# Autodesk Inventor assembly: Motedius_QR-500
(part 2 of 2)
- [Mate]: Motedius_Gelenkfuß_10_PA_M6x60:2 ↔ DIN 125-1 A A 6,4:19
- [Mate]: Motedius_Gelenkfuß_10_PA_M6x60:2 ↔ DIN 125-1 A A 6,4:19
- Einfügen:30 [Insert] (5.5 mm): Motedius_20x20_B-Type_Slot-6_500:2 ↔ DIN 125-1 A A 6,4:19
- [Mate]: Motedius_Gelenkfuß_10_PA_M6x60:3 ↔ DIN 125-1 A A 6,4:20
- [Mate]: Motedius_Gelenkfuß_10_PA_M6x60:3 ↔ DIN 125-1 A A 6,4:20
- [Mate]: Motedius_Gelenkfuß_10_PA_M6x60:4 ↔ DIN 125-1 A A 6,4:21
- [Mate]: Motedius_Gelenkfuß_10_PA_M6x60:4 ↔ DIN 125-1 A A 6,4:21
- Einfügen:31 [Insert] (5.5 mm): Motedius_20x20_B-Type_Slot-6_500:4 ↔ DIN 125-1 A A 6,4:20
- Einfügen:32 [Insert] (5.5 mm): Motedius_20x20_B-Type_Slot-6_500:2 ↔ DIN 125-1 A A 6,4:21
- Passend:88 [Mate]: Motedius_Gelenkfuß_10_PA_M6x60:2 ↔ DIN 125-1 A A 6,4:22
- Passend:89 [Mate]: Motedius_20x20_B-Type_Slot-6_500:1 ↔ DIN 125-1 A A 6,4:22
- Passend:90 [Mate]: Motedius_Gelenkfuß_10_PA_M6x60:4 ↔ DIN 125-1 A A 6,4:23
- Passend:91 [Mate]: Motedius_20x20_B-Type_Slot-6_500:3 ↔ DIN 125-1 A A 6,4:23
- Passend:92 [Mate]: Motedius_Gelenkfuß_10_PA_M6x60:3 ↔ DIN 125-1 A A 6,4:24
- Passend:93 [Mate]: Motedius_20x20_B-Type_Slot-6_500:3 ↔ DIN 125-1 A A 6,4:24
- Passend:94 [Mate]: Motedius_Gelenkfuß_10_PA_M6x60:2 ↔ DIN 934 - ersetzt durch DIN EN 24032/28673/28674 M6:10
- Passend:95 [Mate]: DIN 125-1 A A 6,4:22 ↔ DIN 934 - ersetzt durch DIN EN 24032/28673/28674 M6:10
- Passend:96 [Mate]: Motedius_Gelenkfuß_10_PA_M6x60:4 ↔ DIN 934 - ersetzt durch DIN EN 24032/28673/28674 M6:11
- Passend:97 [Mate]: DIN 125-1 A A 6,4:23 ↔ DIN 934 - ersetzt durch DIN EN 24032/28673/28674 M6:11
- Passend:98 [Mate]: Motedius_Gelenkfuß_10_PA_M6x60:3 ↔ DIN 934 - ersetzt durch DIN EN 24032/28673/28674 M6:12
- Passend:99 [Mate]: DIN 125-1 A A 6,4:24 ↔ DIN 934 - ersetzt durch DIN EN 24032/28673/28674 M6:12
- Passend:135 [Mate]: Motedius_20x20_B-Type_Slot-6_600:1 ↔ Motedius_20x20_B-Type_Slot-6_290:1
- Fluchtend:23 [Flush]: Motedius_20x20_B-Type_Slot-6_600:1 ↔ Motedius_20x20_B-Type_Slot-6_290:1
- Fluchtend:24 [Flush] (290 mm): Motedius_20x20_B-Type_Slot-6_600:1 ↔ Motedius_20x20_B-Type_Slot-6_290:1
- Fluchtend:25 [Flush]: Motedius_20x20_B-Type_Slot-6_600:1 ↔ Motedius_20x20_B-Type_Slot-6_290:2
- Passend:136 [Mate]: Motedius_20x20_B-Type_Slot-6_600:1 ↔ Motedius_20x20_B-Type_Slot-6_290:2
- Fluchtend:26 [Flush] (290 mm): Motedius_20x20_B-Type_Slot-6_600:1 ↔ Motedius_20x20_B-Type_Slot-6_290:2
- Passend:137 [Mate] (30 mm): Motedius_20x20_B-Type_Slot-6_500:3 ↔ Motedius_20x20_B-Type_Slot-6_600:1
- Fluchtend:27 [Flush] (1 mm): Motedius_20x20_B-Type_Slot-6_600:1 ↔ Motedis_Winkel:9
- Passend:138 [Mate]: Motedius_20x20_B-Type_Slot-6_600:1 ↔ Motedis_Winkel:9
- Passend:139 [Mate]: Motedius_20x20_B-Type_Slot-6_290:2 ↔ Motedis_Winkel:9
- Passend:140 [Mate]: Motedius_20x20_B-Type_Slot-6_290:1 ↔ Motedis_Winkel:10
- Passend:141 [Mate]: Motedius_20x20_B-Type_Slot-6_600:1 ↔ Motedis_Winkel:10
- Passend:142 [Mate]: Motedius_20x20_B-Type_Slot-6_600:1 ↔ Motedis_Winkel:11
- Passend:143 [Mate]: Motedius_20x20_B-Type_Slot-6_290:2 ↔ Motedis_Winkel:11
- Fluchtend:28 [Flush] (1 mm): Motedius_20x20_B-Type_Slot-6_290:2 ↔ Motedis_Winkel:11
- Passend:144 [Mate]: Motedius_20x20_B-Type_Slot-6_600:1 ↔ Motedis_Winkel:12
- Passend:145 [Mate]: Motedius_20x20_B-Type_Slot-6_290:1 ↔ Motedis_Winkel:12
- Fluchtend:29 [Flush] (1 mm): Motedius_20x20_B-Type_Slot-6_600:1 ↔ Motedis_Winkel:12
- Fluchtend:31 [Flush] (202.07 mm): Motedius_20x20_B-Type_Slot-6_500:4 ↔ Motedis_Winkel:10
- Passend:159 [Mate] (1.2 mm): Motedius_20x20_B-Type_Slot-6_500_MIR:3 ↔ Mauro_Wagen_QR_version:5
- Passend:160 [Mate] (4.45 mm): Motedius_20x20_B-Type_Slot-6_500_MIR:3 ↔ Mauro_Wagen_QR_version:5
- Passend:161 [Mate] (1.2 mm): Motedius_20x20_B-Type_Slot-6_500_MIR:4 ↔ Mauro_Wagen_QR_version:6
- Passend:162 [Mate] (4.45 mm): Motedius_20x20_B-Type_Slot-6_500_MIR:4 ↔ Mauro_Wagen_QR_version:6
- Passend:163 [Mate] (1.2 mm): Motedius_20x20_B-Type_Slot-6_500_MIR:1 ↔ Mauro_Wagen_QR_version:8
- Passend:164 [Mate] (4.45 mm): Motedius_20x20_B-Type_Slot-6_500_MIR:1 ↔ Mauro_Wagen_QR_version:8
- Passend:165 [Mate] (1.2 mm): Motedius_20x20_B-Type_Slot-6_500_MIR:2 ↔ Mauro_Wagen_QR_version:7
- Passend:166 [Mate] (4.45 mm): Motedius_20x20_B-Type_Slot-6_500_MIR:2 ↔ Mauro_Wagen_QR_version:7
- Fluchtend:32 [Flush]: Mauro_Wagen_QR_version:6 ↔ Mauro_Wagen_QR_version:7
- Fluchtend:33 [Flush]: Mauro_Wagen_QR_version:5 ↔ Mauro_Wagen_QR_version:8
- Einfügen:47 [Insert] (-3 mm): Mauro_Wagen_QR_version:8 ↔ 10mm_Alu_Linearwelle_500mm:1
- Einfügen:48 [Insert] (-3 mm): Mauro_Wagen_QR_version:7 ↔ 10mm_Alu_Linearwelle_500mm:2
- Einfügen:49 [Insert]: Lagerblock_Lm10UU:1 ↔ Linearlager_LM10UU:2
- Einfügen:50 [Insert]: Lagerblock_Lm10UU:1 ↔ Linearlager_LM10UU:1
- Einfügen:51 [Insert] (-200 mm): 10mm_Alu_Linearwelle_500mm:2 ↔ Lagerblock_Lm10UU:1
- Einfügen:52 [Insert] (220 mm): 10mm_Alu_Linearwelle_500mm:1 ↔ Lagerblock_Lm10UU:1
- [Insert] (5.5 mm): Motedius_20x20_B-Type_Slot-6_500:6 ↔ QR_Rahmenschraube_oben_M6x80:2
- [Insert] (5.5 mm): Motedius_20x20_B-Type_Slot-6_500:6 ↔ QR_Rahmenschraube_oben_M6x80:3
- [Insert] (5.5 mm): Motedius_20x20_B-Type_Slot-6_500:5 ↔ QR_Rahmenschraube_oben_M6x80:4
- [Insert] (5.5 mm): Motedius_20x20_B-Type_Slot-6_500:5 ↔ QR_Rahmenschraube_oben_M6x80:5
- [Insert] (5.5 mm): Motedius_20x20_B-Type_Slot-6_500:7 ↔ QR_Rahmenschraube_oben_M6x80:6
- [Insert] (5.5 mm): Motedius_20x20_B-Type_Slot-6_500:7 ↔ QR_Rahmenschraube_oben_M6x80:1
- [Insert] (5.5 mm): Motedius_20x20_B-Type_Slot-6_500:8 ↔ QR_Rahmenschraube_oben_M6x80:7
- [Insert] (5.5 mm): Motedius_20x20_B-Type_Slot-6_500:8 ↔ QR_Rahmenschraube_oben_M6x80:8
- Passend:169 [Mate]: DIN 84 - ersetzt durch DIN EN ISO 1207 M5 x 30:1 ↔ DIN 934 - ersetzt durch DIN EN 24032/28673/28674 M5:2
- Einfügen:65 [Insert] (1 mm): Nema17_Schrittmotor:4 ↔ GT2_20tooth:1
- Einfügen:66 [Insert] (1 mm): Nema17_Schrittmotor:1 ↔ GT2_20tooth:2
- Einfügen:67 [Insert] (1 mm): Nema17_Schrittmotor:2 ↔ GT2_20tooth:3
- Einfügen:68 [Insert] (1 mm): Nema17_Schrittmotor:3 ↔ GT2_20tooth:4
- [Insert] (5.5 mm): Motedius_20x20_B-Type_Slot-6_500:7 ↔ QR_Ramenschraube_unten_M6x60:1
- Einfügen:71 [Insert] (5.5 mm): Motedius_20x20_B-Type_Slot-6_500:5 ↔ QR_Rahmenschraube_oben_M6x80:8
- Einfügen:72 [Insert] (5.5 mm): Motedius_20x20_B-Type_Slot-6_500:5 ↔ QR_Rahmenschraube_oben_M6x80:3
- Einfügen:73 [Insert] (5.5 mm): Motedius_20x20_B-Type_Slot-6_500:8 ↔ QR_Rahmenschraube_oben_M6x80:4
- Einfügen:74 [Insert] (5.5 mm): Motedius_20x20_B-Type_Slot-6_500:8 ↔ QR_Rahmenschraube_oben_M6x80:6
- Einfügen:75 [Insert] (5.5 mm): Motedius_20x20_B-Type_Slot-6_500:7 ↔ QR_Rahmenschraube_oben_M6x80:2
- Einfügen:76 [Insert] (5.5 mm): Motedius_20x20_B-Type_Slot-6_500:6 ↔ QR_Rahmenschraube_oben_M6x80:7
- Einfügen:77 [Insert] (5.5 mm): Motedius_20x20_B-Type_Slot-6_500:6 ↔ QR_Rahmenschraube_oben_M6x80:5
- Einfügen:78 [Insert] (5.5 mm): Motedius_20x20_B-Type_Slot-6_500:7 ↔ QR_Ramenschraube_unten_M6x60:2
- Einfügen:79 [Insert] (5.5 mm): Motedius_20x20_B-Type_Slot-6_500:6 ↔ QR_Ramenschraube_unten_M6x60:4
- Einfügen:80 [Insert] (5.5 mm): Motedius_20x20_B-Type_Slot-6_500:6 ↔ QR_Ramenschraube_unten_M6x60:3
- Einfügen:81 [Insert]: QR_Ramenschraube_unten_M6x60:4 ↔ DIN 9021 6,4:1
- Einfügen:82 [Insert]: DIN 9021 6,4:1 ↔ Distanzscheibe_6x10x0,5mm:1
- Einfügen:83 [Insert]: Seilrolle:1 ↔ Distanzscheibe_6x10x0,5mm:1
- Einfügen:84 [Insert]: Seilrolle:1 ↔ Distanzscheibe_6x10x0,5mm:2
- Einfügen:85 [Insert]: DIN 9021 6,4:2 ↔ Distanzscheibe_6x10x0,5mm:2
- Einfügen:86 [Insert] (5.5 mm): Motedius_20x20_B-Type_Slot-6_500:5 ↔ QR_Ramenschraube_unten_M6x60:6
- Einfügen:87 [Insert] (5.5 mm): Motedius_20x20_B-Type_Slot-6_500:5 ↔ QR_Ramenschraube_unten_M6x60:5
- Einfügen:88 [Insert] (5.5 mm): Motedius_20x20_B-Type_Slot-6_500:8 ↔ QR_Ramenschraube_unten_M6x60:8
- Einfügen:89 [Insert] (5.5 mm): Motedius_20x20_B-Type_Slot-6_500:8 ↔ QR_Ramenschraube_unten_M6x60:7
- [Insert]: Nema17_Schrittmotor:5 ↔ Nema17_Montageplatte_Z-Achse:1
- [Tangent]: Nema17_Schrittmotor:5 ↔ Nema17_Montageplatte_Z-Achse:1
- [Insert] (3 mm): Nema17_Schrittmotor:5 ↔ DIN 84 - ersetzt durch DIN EN ISO 1207 M3 x 6:17
- [Insert] (3 mm): Nema17_Schrittmotor:5 ↔ DIN 84 - ersetzt durch DIN EN ISO 1207 M3 x 6:19
- [Insert] (3 mm): Nema17_Schrittmotor:5 ↔ DIN 84 - ersetzt durch DIN EN ISO 1207 M3 x 6:20
- [Insert] (3 mm): Nema17_Schrittmotor:5 ↔ DIN 84 - ersetzt durch DIN EN ISO 1207 M3 x 6:18
- Passend:175 [Mate] (2.4 mm): Motedius_20x20_B-Type_Slot-6_500_MIR:4 ↔ Nema17_Montageplatte_Z-Achse:1
- Fluchtend:34 [Flush]: Motedius_20x20_B-Type_Slot-6_500_MIR:4 ↔ Nema17_Montageplatte_Z-Achse:1
- Fluchtend:35 [Flush] (45 mm): Motedius_20x20_B-Type_Slot-6_500_MIR:4 ↔ Nema17_Montageplatte_Z-Achse:1
- Einfügen:95 [Insert]: Nema17_Montageplatte_Z-Achse:1 ↔ DIN 9021 5,3:1
- Einfügen:96 [Insert]: DIN 9021 5,3:1 ↔ DIN 9021 5,3:2
- Einfügen:97 [Insert]: Nema17_Montageplatte_Z-Achse:1 ↔ DIN 9021 5,3:4
- Einfügen:98 [Insert]: DIN 9021 5,3:3 ↔ DIN 9021 5,3:4
- Einfügen:99 [Insert] (-8 mm): Nema17_Schrittmotor:5 ↔ Wellenkupplung5-8mm:1
- Einfügen:100 [Insert] (-8 mm): Wellenkupplung5-8mm:1 ↔ Gewindestange_M8x420mm:1
- Passend:176 [Mate]: QR_Ramenschraube_unten_M6x60:4 ↔ DIN 934 - ersetzt durch DIN EN 24032/28673/28674 M6:13
- Passend:177 [Mate]: DIN 9021 6,4:2 ↔ DIN 934 - ersetzt durch DIN EN 24032/28673/28674 M6:13
- [Insert]: DIN 9021 6,4:3 ↔ Distanzscheibe_6x10x0,5mm:3
- [Insert]: Seilrolle:2 ↔ Distanzscheibe_6x10x0,5mm:3
- [Insert]: Seilrolle:2 ↔ Distanzscheibe_6x10x0,5mm:4
- [Insert]: DIN 9021 6,4:4 ↔ Distanzscheibe_6x10x0,5mm:4
- [Mate]: DIN 9021 6,4:4 ↔ DIN 934 - ersetzt durch DIN EN 24032/28673/28674 M6:14
- Einfügen:105 [Insert]: DIN 9021 6,4:4 ↔ DIN 934 - ersetzt durch DIN EN 24032/28673/28674 M6:14
- [Insert]: DIN 9021 6,4:5 ↔ Distanzscheibe_6x10x0,5mm:5
- [Insert]: Seilrolle:3 ↔ Distanzscheibe_6x10x0,5mm:5
- [Insert]: Seilrolle:3 ↔ Distanzscheibe_6x10x0,5mm:6
- [Insert]: DIN 9021 6,4:6 ↔ Distanzscheibe_6x10x0,5mm:6
- [Mate]: DIN 9021 6,4:6 ↔ DIN 934 - ersetzt durch DIN EN 24032/28673/28674 M6:15
- [Insert]: DIN 9021 6,4:6 ↔ DIN 934 - ersetzt durch DIN EN 24032/28673/28674 M6:15
- Einfügen:111 [Insert]: QR_Rahmenschraube_oben_M6x80:5 ↔ DIN 9021 6,4:3
- [Insert]: DIN 9021 6,4:7 ↔ Distanzscheibe_6x10x0,5mm:7
- [Insert]: Seilrolle:4 ↔ Distanzscheibe_6x10x0,5mm:7
- [Insert]: Seilrolle:4 ↔ Distanzscheibe_6x10x0,5mm:8
- [Insert]: DIN 9021 6,4:8 ↔ Distanzscheibe_6x10x0,5mm:8
- [Mate]: DIN 9021 6,4:8 ↔ DIN 934 - ersetzt durch DIN EN 24032/28673/28674 M6:16
- [Insert]: DIN 9021 6,4:8 ↔ DIN 934 - ersetzt durch DIN EN 24032/28673/28674 M6:16
- Einfügen:117 [Insert]: QR_Ramenschraube_unten_M6x60:6 ↔ DIN 9021 6,4:5
- [Insert]: DIN 9021 6,4:9 ↔ Distanzscheibe_6x10x0,5mm:9
- [Insert]: Seilrolle:5 ↔ Distanzscheibe_6x10x0,5mm:9
- [Insert]: Seilrolle:5 ↔ Distanzscheibe_6x10x0,5mm:10
- [Insert]: DIN 9021 6,4:10 ↔ Distanzscheibe_6x10x0,5mm:10
- [Mate]: DIN 9021 6,4:10 ↔ DIN 934 - ersetzt durch DIN EN 24032/28673/28674 M6:17
- [Insert]: DIN 9021 6,4:10 ↔ DIN 934 - ersetzt durch DIN EN 24032/28673/28674 M6:17
- Einfügen:123 [Insert]: QR_Ramenschraube_unten_M6x60:5 ↔ DIN 9021 6,4:7
- [Insert]: DIN 9021 6,4:11 ↔ Distanzscheibe_6x10x0,5mm:11
- [Insert]: Seilrolle:6 ↔ Distanzscheibe_6x10x0,5mm:11
- [Insert]: Seilrolle:6 ↔ Distanzscheibe_6x10x0,5mm:12
- [Insert]: DIN 9021 6,4:12 ↔ Distanzscheibe_6x10x0,5mm:12
- [Mate]: DIN 9021 6,4:12 ↔ DIN 934 - ersetzt durch DIN EN 24032/28673/28674 M6:18
- [Insert]: DIN 9021 6,4:12 ↔ DIN 934 - ersetzt durch DIN EN 24032/28673/28674 M6:18
- Einfügen:129 [Insert]: QR_Ramenschraube_unten_M6x60:7 ↔ DIN 9021 6,4:9
- [Insert]: DIN 9021 6,4:13 ↔ Distanzscheibe_6x10x0,5mm:13
- [Insert]: Seilrolle:7 ↔ Distanzscheibe_6x10x0,5mm:13
- [Insert]: Seilrolle:7 ↔ Distanzscheibe_6x10x0,5mm:14
- [Insert]: DIN 9021 6,4:14 ↔ Distanzscheibe_6x10x0,5mm:14
- [Mate]: DIN 9021 6,4:14 ↔ DIN 934 - ersetzt durch DIN EN 24032/28673/28674 M6:19
- [Insert]: DIN 9021 6,4:14 ↔ DIN 934 - ersetzt durch DIN EN 24032/28673/28674 M6:19
- Einfügen:135 [Insert]: QR_Rahmenschraube_oben_M6x80:6 ↔ DIN 9021 6,4:11
- [Insert]: DIN 9021 6,4:15 ↔ Distanzscheibe_6x10x0,5mm:15
- [Insert]: Seilrolle:8 ↔ Distanzscheibe_6x10x0,5mm:15
- [Insert]: Seilrolle:8 ↔ Distanzscheibe_6x10x0,5mm:16
- [Insert]: DIN 9021 6,4:16 ↔ Distanzscheibe_6x10x0,5mm:16
- [Mate]: DIN 9021 6,4:16 ↔ DIN 934 - ersetzt durch DIN EN 24032/28673/28674 M6:20
- [Insert]: DIN 9021 6,4:16 ↔ DIN 934 - ersetzt durch DIN EN 24032/28673/28674 M6:20
- Einfügen:141 [Insert]: QR_Ramenschraube_unten_M6x60:8 ↔ DIN 9021 6,4:13
- [Insert]: DIN 9021 6,4:17 ↔ Distanzscheibe_6x10x0,5mm:17
- [Insert]: Seilrolle:9 ↔ Distanzscheibe_6x10x0,5mm:17
- [Insert]: Seilrolle:9 ↔ Distanzscheibe_6x10x0,5mm:18
- [Insert]: DIN 9021 6,4:18 ↔ Distanzscheibe_6x10x0,5mm:18
- [Mate]: DIN 9021 6,4:18 ↔ DIN 934 - ersetzt durch DIN EN 24032/28673/28674 M6:21
- [Insert]: DIN 9021 6,4:18 ↔ DIN 934 - ersetzt durch DIN EN 24032/28673/28674 M6:21
- Einfügen:147 [Insert]: QR_Ramenschraube_unten_M6x60:1 ↔ DIN 9021 6,4:15
- Einfügen:148 [Insert]: QR_Rahmenschraube_oben_M6x80:1 ↔ DIN 9021 6,4:17
- Passend:186 [Mate]: Motedius_20x20_B-Type_Slot-6_290:1 ↔ Z-Stage_Wheel_plate:1
- Fluchtend:36 [Flush]: Motedius_20x20_B-Type_Slot-6_290:1 ↔ Z-Stage_Wheel_plate:1
- Fluchtend:37 [Flush] (-22.2 mm): Motedius_20x20_B-Type_Slot-6_290:1 ↔ Z-Stage_Wheel_plate:1
- Passend:187 [Mate]: Motedius_20x20_B-Type_Slot-6_290:1 ↔ Z-Stage_Wheel_plate:2
- Fluchtend:38 [Flush]: Motedius_20x20_B-Type_Slot-6_290:1 ↔ Z-Stage_Wheel_plate:2
- Fluchtend:39 [Flush] (-22.2 mm): Motedius_20x20_B-Type_Slot-6_290:1 ↔ Z-Stage_Wheel_plate:2
- Einfügen:149 [Insert] (-51.5 mm): Gewindestück_M5_Z-Achse:1 ↔ Z-Stage_Wheel_plate:1
- Einfügen:150 [Insert] (4.55 mm): Openbuilds_Dual_V-Wheel:8 ↔ Z-Stage_Wheel_plate:1
- Passend:188 [Mate]: Gewindestück_M5_Z-Achse:1 ↔ DIN 934 - ersetzt durch DIN EN 24032/28673/28674 M5:5
- Passend:189 [Mate]: Z-Stage_Wheel_plate:1 ↔ DIN 934 - ersetzt durch DIN EN 24032/28673/28674 M5:5
- Passend:190 [Mate]: Gewindestück_M5_Z-Achse:1 ↔ DIN 934 - ersetzt durch DIN EN 24032/28673/28674 M5:6
- Passend:191 [Mate]: Z-Stage_Wheel_plate:2 ↔ DIN 934 - ersetzt durch DIN EN 24032/28673/28674 M5:6
- Passend:192 [Mate]: Gewindestück_M5_Z-Achse:1 ↔ DIN 934 - ersetzt durch DIN EN 24032/28673/28674 M5:7
- Passend:193 [Mate]: Z-Stage_Wheel_plate:1 ↔ DIN 934 - ersetzt durch DIN EN 24032/28673/28674 M5:7
- Passend:194 [Mate]: Gewindestück_M5_Z-Achse:1 ↔ DIN 934 - ersetzt durch DIN EN 24032/28673/28674 M5:8
- Passend:195 [Mate]: Z-Stage_Wheel_plate:2 ↔ DIN 934 - ersetzt durch DIN EN 24032/28673/28674 M5:8
- Passend:196 [Mate]: Motedius_20x20_B-Type_Slot-6_600:1 ↔ Z-Stage_Wheel_plate_20x20:2
- Fluchtend:40 [Flush]: Motedius_20x20_B-Type_Slot-6_600:1 ↔ Z-Stage_Wheel_plate_20x20:2
- Fluchtend:41 [Flush] (-22.2 mm): Motedius_20x20_B-Type_Slot-6_600:1 ↔ Z-Stage_Wheel_plate_20x20:2
- Fluchtend:42 [Flush]: Motedius_20x20_B-Type_Slot-6_600:1 ↔ Z-Stage_Wheel_plate_20x20:1
- Passend:197 [Mate]: Motedius_20x20_B-Type_Slot-6_600:1 ↔ Z-Stage_Wheel_plate_20x20:1
- Fluchtend:43 [Flush]: Z-Stage_Wheel_plate_20x20:1 ↔ Z-Stage_Wheel_plate_20x20:2
- Einfügen:151 [Insert]: DIN 84 - ersetzt durch DIN EN ISO 1207 M5 x 30:1 ↔ Z-Stage_Wheel_plate_20x20:2
- Einfügen:152 [Insert]: DIN 934 - ersetzt durch DIN EN 24032/28673/28674 M5:2 ↔ Z-Stage_Wheel_plate_20x20:1
- Fluchtend:44 [Flush] (201.008 mm): Motedius_20x20_B-Type_Slot-6_500:2 ↔ Motedis_Winkel:11
- Fluchtend:45 [Flush] (201.008 mm): Motedius_20x20_B-Type_Slot-6_500:3 ↔ Motedis_Winkel:9
- Einfügen:153 [Insert] (4.55 mm): Openbuilds_Dual_V-Wheel:6 ↔ Z-Stage_Wheel_plate_20x20:2
- Passend:198 [Mate]: DIN 84 - ersetzt durch DIN EN ISO 1207 M5 x 30:1 ↔ DIN 934 - ersetzt durch DIN EN 24032/28673/28674 M5:9
- Passend:199 [Mate]: Z-Stage_Wheel_plate_20x20:2 ↔ DIN 934 - ersetzt durch DIN EN 24032/28673/28674 M5:9
- Passend:200 [Mate]: DIN 84 - ersetzt durch DIN EN ISO 1207 M5 x 30:1 ↔ DIN 934 - ersetzt durch DIN EN 24032/28673/28674 M5:10
- Passend:201 [Mate]: Z-Stage_Wheel_plate_20x20:1 ↔ DIN 934 - ersetzt durch DIN EN 24032/28673/28674 M5:10
- Passend:202 [Mate]: Motedius_20x20_B-Type_Slot-6_600:1 ↔ Z-Stage_Wheel_plate_20x20:3
- Fluchtend:46 [Flush]: Motedius_20x20_B-Type_Slot-6_600:1 ↔ Z-Stage_Wheel_plate_20x20:3
- Fluchtend:47 [Flush] (-22.2 mm): Motedius_20x20_B-Type_Slot-6_600:1 ↔ Z-Stage_Wheel_plate_20x20:3
- Passend:203 [Mate]: Motedius_20x20_B-Type_Slot-6_600:1 ↔ Z-Stage_Wheel_plate:3
- Fluchtend:48 [Flush]: Motedius_20x20_B-Type_Slot-6_600:1 ↔ Z-Stage_Wheel_plate:3
- Fluchtend:49 [Flush]: Z-Stage_Wheel_plate_20x20:3 ↔ Z-Stage_Wheel_plate:3
- [Insert]: Z-Stage_Wheel_plate_20x20:3 ↔ Gewindestück_M5_Z-Achse_55mm:1
- Einfügen:155 [Insert] (4.55 mm): Openbuilds_Dual_V-Wheel:5 ↔ Z-Stage_Wheel_plate:3
- [Mate]: Gewindestück_M5_Z-Achse_55mm:1 ↔ DIN 934 - ersetzt durch DIN EN 24032/28673/28674 M5:11
- Passend:205 [Mate]: Z-Stage_Wheel_plate_20x20:3 ↔ DIN 934 - ersetzt durch DIN EN 24032/28673/28674 M5:11
- [Mate]: Gewindestück_M5_Z-Achse_55mm:1 ↔ DIN 934 - ersetzt durch DIN EN 24032/28673/28674 M5:12
- Passend:207 [Mate]: Z-Stage_Wheel_plate:3 ↔ DIN 934 - ersetzt durch DIN EN 24032/28673/28674 M5:12
- [Mate]: Gewindestück_M5_Z-Achse_55mm:1 ↔ DIN 934 - ersetzt durch DIN EN 24032/28673/28674 M5:13
- Passend:209 [Mate]: Z-Stage_Wheel_plate:3 ↔ DIN 934 - ersetzt durch DIN EN 24032/28673/28674 M5:13
- Fluchtend:50 [Flush]: Motedius_20x20_B-Type_Slot-6_290:2 ↔ Z-Stage_Wheel_plate_20x20:4
- Passend:210 [Mate]: Motedius_20x20_B-Type_Slot-6_290:2 ↔ Z-Stage_Wheel_plate_20x20:4
- Fluchtend:51 [Flush] (-22.2 mm): Motedius_20x20_B-Type_Slot-6_290:2 ↔ Z-Stage_Wheel_plate_20x20:4
- Passend:211 [Mate]: Motedius_20x20_B-Type_Slot-6_290:2 ↔ Z-Stage_Wheel_plate_20x20:5
- Fluchtend:52 [Flush]: Motedius_20x20_B-Type_Slot-6_290:2 ↔ Z-Stage_Wheel_plate_20x20:5
- Fluchtend:53 [Flush]: Z-Stage_Wheel_plate_20x20:4 ↔ Z-Stage_Wheel_plate_20x20:5
- Einfügen:156 [Insert]: DIN 84 - ersetzt durch DIN EN ISO 1207 M5 x 30:2 ↔ Z-Stage_Wheel_plate_20x20:4
- Passend:212 [Mate]: DIN 84 - ersetzt durch DIN EN ISO 1207 M5 x 30:2 ↔ DIN 934 - ersetzt durch DIN EN 24032/28673/28674 M5:14
- Passend:213 [Mate]: Z-Stage_Wheel_plate_20x20:5 ↔ DIN 934 - ersetzt durch DIN EN 24032/28673/28674 M5:14
- Einfügen:157 [Insert] (4.55 mm): Openbuilds_Dual_V-Wheel:7 ↔ Z-Stage_Wheel_plate_20x20:4
- Passend:214 [Mate]: DIN 84 - ersetzt durch DIN EN ISO 1207 M5 x 30:2 ↔ DIN 934 - ersetzt durch DIN EN 24032/28673/28674 M5:15
- Passend:215 [Mate]: Z-Stage_Wheel_plate_20x20:4 ↔ DIN 934 - ersetzt durch DIN EN 24032/28673/28674 M5:15
- Passend:216 [Mate]: DIN 84 - ersetzt durch DIN EN ISO 1207 M5 x 30:2 ↔ DIN 934 - ersetzt durch DIN EN 24032/28673/28674 M5:16
- Passend:217 [Mate]: Z-Stage_Wheel_plate_20x20:5 ↔ DIN 934 - ersetzt durch DIN EN 24032/28673/28674 M5:16
- Einfügen:158 [Insert] (-5 mm): Z-Stage_Wheel_plate_20x20:2 ↔ Ösenschraube_M3x15:1
- Passend:218 [Mate]: Ösenschraube_M3x15:1 ↔ DIN 934 - ersetzt durch DIN EN 24032/28673/28674 M3:1
- Passend:219 [Mate]: Z-Stage_Wheel_plate_20x20:2 ↔ DIN 934 - ersetzt durch DIN EN 24032/28673/28674 M3:1
- Passend:220 [Mate]: Ösenschraube_M3x15:1 ↔ DIN 934 - ersetzt durch DIN EN 24032/28673/28674 M3:2
- Passend:221 [Mate]: Z-Stage_Wheel_plate_20x20:2 ↔ DIN 934 - ersetzt durch DIN EN 24032/28673/28674 M3:2
- Einfügen:159 [Insert] (-5 mm): Z-Stage_Wheel_plate_20x20:3 ↔ Ösenschraube_M3x15:2
- Einfügen:160 [Insert] (-5 mm): Z-Stage_Wheel_plate_20x20:4 ↔ Ösenschraube_M3x15:3
- Passend:222 [Mate]: Ösenschraube_M3x15:3 ↔ DIN 934 - ersetzt durch DIN EN 24032/28673/28674 M3:3
- Passend:223 [Mate]: Z-Stage_Wheel_plate_20x20:4 ↔ DIN 934 - ersetzt durch DIN EN 24032/28673/28674 M3:3
- Passend:224 [Mate]: Ösenschraube_M3x15:3 ↔ DIN 934 - ersetzt durch DIN EN 24032/28673/28674 M3:4
- Passend:225 [Mate]: Z-Stage_Wheel_plate_20x20:4 ↔ DIN 934 - ersetzt durch DIN EN 24032/28673/28674 M3:4
- Passend:226 [Mate]: Ösenschraube_M3x15:2 ↔ DIN 934 - ersetzt durch DIN EN 24032/28673/28674 M3:5
- Passend:227 [Mate]: Z-Stage_Wheel_plate_20x20:3 ↔ DIN 934 - ersetzt durch DIN EN 24032/28673/28674 M3:5
- Passend:228 [Mate]: Ösenschraube_M3x15:2 ↔ DIN 934 - ersetzt durch DIN EN 24032/28673/28674 M3:6
- Passend:229 [Mate]: Z-Stage_Wheel_plate_20x20:3 ↔ DIN 934 - ersetzt durch DIN EN 24032/28673/28674 M3:6
- Einfügen:161 [Insert]: Z-Stage_Wheel_plate_20x20:3 ↔ DIN 84 - ersetzt durch DIN EN ISO 1207 M5 x 6:1
- Einfügen:162 [Insert]: Z-Stage_Wheel_plate_20x20:3 ↔ DIN 84 - ersetzt durch DIN EN ISO 1207 M5 x 6:2
- Einfügen:163 [Insert]: Z-Stage_Wheel_plate_20x20:5 ↔ DIN 84 - ersetzt durch DIN EN ISO 1207 M5 x 6:4
- Einfügen:164 [Insert]: Z-Stage_Wheel_plate_20x20:5 ↔ DIN 84 - ersetzt durch DIN EN ISO 1207 M5 x 6:3
- Einfügen:165 [Insert]: Z-Stage_Wheel_plate_20x20:4 ↔ DIN 84 - ersetzt durch DIN EN ISO 1207 M5 x 6:5
- Einfügen:166 [Insert]: Z-Stage_Wheel_plate_20x20:4 ↔ DIN 84 - ersetzt durch DIN EN ISO 1207 M5 x 6:6
- Einfügen:167 [Insert]: Z-Stage_Wheel_plate_20x20:2 ↔ DIN 84 - ersetzt durch DIN EN ISO 1207 M5 x 6:7
- Einfügen:168 [Insert]: Z-Stage_Wheel_plate_20x20:2 ↔ DIN 84 - ersetzt durch DIN EN ISO 1207 M5 x 6:8
- Einfügen:169 [Insert]: Z-Stage_Wheel_plate_20x20:1 ↔ DIN 84 - ersetzt durch DIN EN ISO 1207 M5 x 6:9
- Einfügen:170 [Insert]: Z-Stage_Wheel_plate_20x20:1 ↔ DIN 84 - ersetzt durch DIN EN ISO 1207 M5 x 6:10
- Einfügen:171 [Insert]: Z-Stage_Wheel_plate:2 ↔ DIN 84 - ersetzt durch DIN EN ISO 1207 M5 x 6:11
- Einfügen:172 [Insert]: Z-Stage_Wheel_plate:2 ↔ DIN 84 - ersetzt durch DIN EN ISO 1207 M5 x 6:12
- Einfügen:173 [Insert]: Z-Stage_Wheel_plate:1 ↔ DIN 84 - ersetzt durch DIN EN ISO 1207 M5 x 6:13
- Einfügen:174 [Insert]: Z-Stage_Wheel_plate:1 ↔ DIN 84 - ersetzt durch DIN EN ISO 1207 M5 x 6:14
- Einfügen:175 [Insert]: Z-Stage_Wheel_plate:3 ↔ DIN 84 - ersetzt durch DIN EN ISO 1207 M5 x 6:15
- Einfügen:176 [Insert]: Z-Stage_Wheel_plate:3 ↔ DIN 84 - ersetzt durch DIN EN ISO 1207 M5 x 6:16
- Einfügen:177 [Insert]: Motedis_Winkel:10 ↔ DIN 84 - ersetzt durch DIN EN ISO 1207 M5 x 8:2
- Einfügen:178 [Insert]: Motedis_Winkel:10 ↔ DIN 84 - ersetzt durch DIN EN ISO 1207 M5 x 8:1
- Einfügen:179 [Insert]: Motedis_Winkel:9 ↔ DIN 84 - ersetzt durch DIN EN ISO 1207 M5 x 8:3
- Einfügen:180 [Insert]: Motedis_Winkel:9 ↔ DIN 84 - ersetzt durch DIN EN ISO 1207 M5 x 8:4
- Einfügen:181 [Insert]: Motedis_Winkel:11 ↔ DIN 84 - ersetzt durch DIN EN ISO 1207 M5 x 8:5
- Einfügen:182 [Insert]: Motedis_Winkel:11 ↔ DIN 84 - ersetzt durch DIN EN ISO 1207 M5 x 8:6
- Einfügen:183 [Insert]: Motedis_Winkel:12 ↔ DIN 84 - ersetzt durch DIN EN ISO 1207 M5 x 8:7
- Einfügen:184 [Insert]: Motedis_Winkel:12 ↔ DIN 84 - ersetzt durch DIN EN ISO 1207 M5 x 8:8
- Einfügen:185 [Insert]: DIN 934 - ersetzt durch DIN EN 24032/28673/28674 M8:1 ↔ Z_Stage_Nut_holder_15x15alu:1
- Passend:230 [Mate]: DIN 934 - ersetzt durch DIN EN 24032/28673/28674 M8:1 ↔ Z_Stage_Nut_holder_15x15alu:1
- Einfügen:186 [Insert]: Z_Stage_Nut_holder_15x15alu:1 ↔ DIN 934 - ersetzt durch DIN EN 24032/28673/28674 M8:2
- Passend:231 [Mate]: Z_Stage_Nut_holder_15x15alu:1 ↔ DIN 934 - ersetzt durch DIN EN 24032/28673/28674 M8:2
- Passend:232 [Mate]: Motedius_20x20_B-Type_Slot-6_290:1 ↔ Z_Stage_Nut_holder_15x15alu:1
- Tangential:12: Gewindestange_M8x420mm:1 ↔ DIN 934 - ersetzt durch DIN EN 24032/28673/28674 M8:1
- Passend:233 [Mate]: DIN 84 - ersetzt durch DIN EN ISO 1207 M5 x 20:1 ↔ DIN 9021 5,3:5
- Passend:234 [Mate]: DIN 84 - ersetzt durch DIN EN ISO 1207 M5 x 20:1 ↔ DIN 9021 5,3:5
- Einfügen:187 [Insert]: Z_Stage_Nut_holder_15x15alu:1 ↔ DIN 9021 5,3:5
- Einfügen:188 [Insert]: Aluplatte_5mm:1 ↔ DIN 84 - ersetzt durch DIN EN ISO 1207 M5 x 40:3
- Einfügen:189 [Insert]: Aluplatte_5mm:1 ↔ DIN 84 - ersetzt durch DIN EN ISO 1207 M5 x 40:2
- Einfügen:190 [Insert]: Aluplatte_5mm:1 ↔ DIN 84 - ersetzt durch DIN EN ISO 1207 M5 x 40:4
- Einfügen:191 [Insert]: Aluplatte_5mm:1 ↔ DIN 84 - ersetzt durch DIN EN ISO 1207 M5 x 40:5
- Fluchtend:54 [Flush] (40 mm): Motedius_20x20_B-Type_Slot-6_500:4 ↔ Aluplatte_5mm:1
- Fluchtend:55 [Flush] (40 mm): Motedius_20x20_B-Type_Slot-6_500:1 ↔ Aluplatte_5mm:1
- Passend:235 [Mate]: Motedius_20x20_B-Type_Slot-6_600:1 ↔ DIN 84 - ersetzt durch DIN EN ISO 1207 M5 x 40:3
- Passend:236 [Mate]: DIN 84 - ersetzt durch DIN EN ISO 1207 M5 x 40:3 ↔ DIN 9021 5,3:6
- Passend:237 [Mate]: Motedius_20x20_B-Type_Slot-6_600:1 ↔ DIN 9021 5,3:6
- Passend:238 [Mate]: DIN 84 - ersetzt durch DIN EN ISO 1207 M5 x 40:2 ↔ DIN 9021 5,3:7
- Passend:239 [Mate]: Motedius_20x20_B-Type_Slot-6_290:2 ↔ DIN 9021 5,3:7
- Passend:240 [Mate]: DIN 84 - ersetzt durch DIN EN ISO 1207 M5 x 40:4 ↔ DIN 9021 5,3:8
- Passend:241 [Mate]: Motedius_20x20_B-Type_Slot-6_290:1 ↔ DIN 9021 5,3:8
- Passend:242 [Mate]: DIN 84 - ersetzt durch DIN EN ISO 1207 M5 x 40:5 ↔ DIN 9021 5,3:9
- Passend:243 [Mate]: Motedius_20x20_B-Type_Slot-6_600:1 ↔ DIN 9021 5,3:9
- Passend:244 [Mate]: DIN 84 - ersetzt durch DIN EN ISO 1207 M5 x 40:3 ↔ DIN 934 - ersetzt durch DIN EN 24032/28673/28674 M5:17
- Passend:245 [Mate]: DIN 9021 5,3:6 ↔ DIN 934 - ersetzt durch DIN EN 24032/28673/28674 M5:17
- Passend:246 [Mate]: DIN 84 - ersetzt durch DIN EN ISO 1207 M5 x 40:5 ↔ DIN 934 - ersetzt durch DIN EN 24032/28673/28674 M5:18
- Passend:247 [Mate]: DIN 9021 5,3:9 ↔ DIN 934 - ersetzt durch DIN EN 24032/28673/28674 M5:18
- Passend:248 [Mate]: DIN 84 - ersetzt durch DIN EN ISO 1207 M5 x 40:4 ↔ DIN 934 - ersetzt durch DIN EN 24032/28673/28674 M5:19
- Passend:249 [Mate]: DIN 9021 5,3:8 ↔ DIN 934 - ersetzt durch DIN EN 24032/28673/28674 M5:19
- Passend:250 [Mate]: DIN 84 - ersetzt durch DIN EN ISO 1207 M5 x 40:2 ↔ DIN 934 - ersetzt durch DIN EN 24032/28673/28674 M5:20
- Passend:251 [Mate]: DIN 9021 5,3:7 ↔ DIN 934 - ersetzt durch DIN EN 24032/28673/28674 M5:20
- Passend:252 [Mate]: DIN 84 - ersetzt durch DIN EN ISO 1207 M5 x 40:4 ↔ DIN 934 - ersetzt durch DIN EN 24032/28673/28674 M5:21
- Passend:253 [Mate]: Aluplatte_5mm:1 ↔ DIN 934 - ersetzt durch DIN EN 24032/28673/28674 M5:21
- Passend:254 [Mate]: DIN 84 - ersetzt durch DIN EN ISO 1207 M5 x 40:5 ↔ DIN 934 - ersetzt durch DIN EN 24032/28673/28674 M5:22
- Passend:255 [Mate]: Aluplatte_5mm:1 ↔ DIN 934 - ersetzt durch DIN EN 24032/28673/28674 M5:22
- Passend:256 [Mate]: DIN 84 - ersetzt durch DIN EN ISO 1207 M5 x 40:2 ↔ DIN 934 - ersetzt durch DIN EN 24032/28673/28674 M5:23
- Passend:257 [Mate]: Aluplatte_5mm:1 ↔ DIN 934 - ersetzt durch DIN EN 24032/28673/28674 M5:23
- Passend:258 [Mate]: DIN 84 - ersetzt durch DIN EN ISO 1207 M5 x 40:3 ↔ DIN 934 - ersetzt durch DIN EN 24032/28673/28674 M5:24
- Passend:259 [Mate]: Aluplatte_5mm:1 ↔ DIN 934 - ersetzt durch DIN EN 24032/28673/28674 M5:24
- Fluchtend:56 [Flush] (-2.5 mm): Seilrolle:4
- Fluchtend:57 [Flush]: Seil2:1
- Fluchtend:58 [Flush]: Seil2:1
- Fluchtend:59 [Flush] (-2.5 mm): Seilrolle:7
- Fluchtend:60 [Flush]: Seil-3:1
- Fluchtend:61 [Flush]: Seil-3:1
- Einfügen:192 [Insert] (-4 mm): Z-Stage_Wheel_plate_20x20:3 ↔ Gewindestück_M5_Z-Achse_55mm:1
- Passend:260 [Mate]: Gewindestück_M5_Z-Achse_55mm:1 ↔ DIN 934 - ersetzt durch DIN EN 24032/28673/28674 M5:25
- Passend:261 [Mate]: Z-Stage_Wheel_plate_20x20:3 ↔ DIN 934 - ersetzt durch DIN EN 24032/28673/28674 M5:25
- Passend:262 [Mate]: Motedius_20x20_B-Type_Slot-6_500_MIR:2 ↔ Motedius_20x20_B-Type_Slot-6_120:1
- Fluchtend:62 [Flush]: Motedius_20x20_B-Type_Slot-6_500_MIR:2 ↔ Motedius_20x20_B-Type_Slot-6_120:1
- Passend:263 [Mate] (-40 mm): Motedius_20x20_B-Type_Slot-6_500_MIR:2 ↔ Motedius_20x20_B-Type_Slot-6_120:1
- Passend:264 [Mate]: Motedius_20x20_B-Type_Slot-6_120:1 ↔ extruder_180Grad:1
- Fluchtend:63 [Flush]: Motedius_20x20_B-Type_Slot-6_120:1 ↔ extruder_180Grad:1
- Fluchtend:64 [Flush]: Motedius_20x20_B-Type_Slot-6_120:1 ↔ extruder_180Grad:1
- Passend:265 [Mate]: DIN 84 - M6 x 70:1 ↔ DIN 9021 6,4:19
- Passend:266 [Mate]: Motedius_20x20_B-Type_Slot-6_120:1 ↔ DIN 9021 6,4:19
- Passend:267 [Mate]: DIN 84 - M6 x 70:1 ↔ DIN 934 - ersetzt durch DIN EN 24032/28673/28674 M6:22
- Passend:268 [Mate]: DIN 9021 6,4:19 ↔ DIN 934 - ersetzt durch DIN EN 24032/28673/28674 M6:22
- Einfügen:193 [Insert]: Nema17_Montageplatte_Z-Achse:1 ↔ DIN 84 - ersetzt durch DIN EN ISO 1207 M5 x 10:1
- Einfügen:194 [Insert]: Nema17_Montageplatte_Z-Achse:1 ↔ DIN 84 - ersetzt durch DIN EN ISO 1207 M5 x 10:2
- Einfügen:195 [Insert]: Lagerblock_Lm10UU:1 ↔ E3D_V6_1.75mm_Universal_HotEnd_Mockup:1
- Tangential:13: E3D_V6_1.75mm_Universal_HotEnd_Mockup:1 ↔ E3D_V6_Fan_Duct:1
- Passend:269 [Mate]: E3D_V6_1.75mm_Universal_HotEnd_Mockup:1
- Passend:270 [Mate]: extruder_180Grad:1
- Passend:271 [Mate]
- Passend:272 [Mate]
- Fluchtend:65 [Flush]: PTFE_Tube_4x2:1
- Fluchtend:66 [Flush]: E3D_V6_1.75mm_Universal_HotEnd_Mockup:1 ↔ PTFE_Tube_4x2:1
- Einfügen:196 [Insert]: E3D_V6_Fan_Duct:1 ↔ 12VDC-1.1875-X-0.375-DELTA-BOX-FAN:1
- Einfügen:197 [Insert]: Lagerblock_Lm10UU:1 ↔ DIN 84 - ersetzt durch DIN EN ISO 1207 M3 x 10:1
- Einfügen:198 [Insert]: Lagerblock_Lm10UU:1 ↔ DIN 84 - ersetzt durch DIN EN ISO 1207 M3 x 10:2
- Passend:273 [Mate]: DIN 84 - ersetzt durch DIN EN ISO 1207 M3 x 10:1 ↔ DIN 934 - ersetzt durch DIN EN 24032/28673/28674 M3:7
- Passend:274 [Mate]: Lagerblock_Lm10UU:1 ↔ DIN 934 - ersetzt durch DIN EN 24032/28673/28674 M3:7
- Passend:275 [Mate]: DIN 84 - ersetzt durch DIN EN ISO 1207 M3 x 10:2 ↔ DIN 934 - ersetzt durch DIN EN 24032/28673/28674 M3:8
- Passend:276 [Mate]: Lagerblock_Lm10UU:1 ↔ DIN 934 - ersetzt durch DIN EN 24032/28673/28674 M3:8
- Einfügen:199 [Insert]: Lagerblock_Lm10UU:1 ↔ DIN 84 - ersetzt durch DIN EN ISO 1207 M3 x 22:2
- Einfügen:200 [Insert]: Lagerblock_Lm10UU:1 ↔ DIN 84 - ersetzt durch DIN EN ISO 1207 M3 x 22:1
- Passend:277 [Mate]: DIN 84 - ersetzt durch DIN EN ISO 1207 M3 x 22:1 ↔ DIN 934 - ersetzt durch DIN EN 24032/28673/28674 M3:9
- Passend:278 [Mate]: Lagerblock_Lm10UU:1 ↔ DIN 934 - ersetzt durch DIN EN 24032/28673/28674 M3:9
- Passend:279 [Mate]: DIN 84 - ersetzt durch DIN EN ISO 1207 M3 x 22:2 ↔ DIN 934 - ersetzt durch DIN EN 24032/28673/28674 M3:10
- Passend:280 [Mate]: Lagerblock_Lm10UU:1 ↔ DIN 934 - ersetzt durch DIN EN 24032/28673/28674 M3:10
- Einfügen:201 [Insert]: Lagerblock_Lm10UU:1 ↔ DIN 84 - ersetzt durch DIN EN ISO 1207 M3 x 18:2
- Einfügen:202 [Insert]: Lagerblock_Lm10UU:1 ↔ DIN 84 - ersetzt durch DIN EN ISO 1207 M3 x 18:1
- Passend:281 [Mate]: DIN 84 - ersetzt durch DIN EN ISO 1207 M3 x 18:2 ↔ DIN 934 - ersetzt durch DIN EN 24032/28673/28674 M3:11
- Passend:282 [Mate]: Lagerblock_Lm10UU:1 ↔ DIN 934 - ersetzt durch DIN EN 24032/28673/28674 M3:11
- Passend:283 [Mate]: DIN 84 - ersetzt durch DIN EN ISO 1207 M3 x 18:1 ↔ DIN 934 - ersetzt durch DIN EN 24032/28673/28674 M3:12
- Passend:284 [Mate]: Lagerblock_Lm10UU:1 ↔ DIN 934 - ersetzt durch DIN EN 24032/28673/28674 M3:12
- Passend:285 [Mate] (0.5 mm): Mauro_Wagen_QR_version:8 ↔ gt2_clip_v2:1
- Fluchtend:67 [Flush]: Mauro_Wagen_QR_version:8 ↔ gt2_clip_v2:1
- Fluchtend:68 [Flush] (0.5 mm): Mauro_Wagen_QR_version:8 ↔ gt2_clip_v2:1
- Passend:286 [Mate]: Mauro_Wagen_QR_version:8 ↔ gt2_clip_v2:1
- Passend:287 [Mate]: Mauro_Wagen_QR_version:6 ↔ gt2_clip_v2:4
- Fluchtend:69 [Flush]: Mauro_Wagen_QR_version:6 ↔ gt2_clip_v2:4
- Fluchtend:70 [Flush] (0.5 mm): Mauro_Wagen_QR_version:6 ↔ gt2_clip_v2:4
- Passend:288 [Mate]: Mauro_Wagen_QR_version:7 ↔ gt2_clip_v2:3
- Fluchtend:71 [Flush]: Mauro_Wagen_QR_version:7 ↔ gt2_clip_v2:3
- Fluchtend:72 [Flush] (0.5 mm): Mauro_Wagen_QR_version:7 ↔ gt2_clip_v2:3
- Passend:289 [Mate]: Mauro_Wagen_QR_version:5 ↔ gt2_clip_v2:2
- Fluchtend:73 [Flush]: Mauro_Wagen_QR_version:5 ↔ gt2_clip_v2:2
- Fluchtend:74 [Flush] (0.5 mm): Mauro_Wagen_QR_version:5 ↔ gt2_clip_v2:2
- Einfügen:203 [Insert]: Mauro_Wagen_QR_version:5 ↔ DIN 84 - ersetzt durch DIN EN ISO 1207 M3 x 14:1
- Einfügen:204 [Insert]: Mauro_Wagen_QR_version:6 ↔ DIN 84 - ersetzt durch DIN EN ISO 1207 M3 x 14:2
- Einfügen:205 [Insert]: Mauro_Wagen_QR_version:8 ↔ DIN 84 - ersetzt durch DIN EN ISO 1207 M3 x 14:3
- Einfügen:206 [Insert]: Mauro_Wagen_QR_version:7 ↔ DIN 84 - ersetzt durch DIN EN ISO 1207 M3 x 14:4
- Passend:290 [Mate]: DIN 84 - ersetzt durch DIN EN ISO 1207 M3 x 14:1 ↔ DIN 934 - ersetzt durch DIN EN 24032/28673/28674 M3:13
- Passend:291 [Mate]: gt2_clip_v2:2 ↔ DIN 934 - ersetzt durch DIN EN 24032/28673/28674 M3:13
- Passend:292 [Mate]: DIN 84 - ersetzt durch DIN EN ISO 1207 M3 x 14:2 ↔ DIN 934 - ersetzt durch DIN EN 24032/28673/28674 M3:14
- Passend:293 [Mate]: gt2_clip_v2:4 ↔ DIN 934 - ersetzt durch DIN EN 24032/28673/28674 M3:14
- Passend:294 [Mate]: DIN 84 - ersetzt durch DIN EN ISO 1207 M3 x 14:3 ↔ DIN 934 - ersetzt durch DIN EN 24032/28673/28674 M3:15
- Passend:295 [Mate]: gt2_clip_v2:1 ↔ DIN 934 - ersetzt durch DIN EN 24032/28673/28674 M3:15
- Passend:296 [Mate]: DIN 84 - ersetzt durch DIN EN ISO 1207 M3 x 14:4 ↔ DIN 934 - ersetzt durch DIN EN 24032/28673/28674 M3:16
- Passend:297 [Mate]: gt2_clip_v2:3 ↔ DIN 934 - ersetzt durch DIN EN 24032/28673/28674 M3:16
## Named parameters: d90_d82 = 3 mm, d91_d83 = 3 mm, d92_d84 = 3 mm, d93_d85 = 3 mm, d94_d79 = 0 mm, d95_d80 = 0 mm, d99_d90_d82 = 3 mm, d100_d91_d83 = 3 mm, d101_d92_d84 = 3 mm, d102_d93_d85 = 3 mm, d103_d94_d79 = 0 mm, d104_d95_d80 = 0 mm, d108_d99_d90_d82 = 3 mm, d109_d100_d91_d83 = 3 mm, d110_d101_d92_d84 = 3 mm, d111_d102_d93_d85 = 3 mm, d112_d103_d94_d79 = 0 mm, d113_d104_d95_d80 = 0 mm, d163_d161 = 0 mm, d164_d162 = 0 mm, d165_d161 = 0 mm, d166_d162 = 0 mm, d167_d161 = 0 mm, d168_d162 = 0 mm, d196_d190 = 0 mm, d200_d189 = 0 mm, d202_d196_d190 = 0 mm, d203_d200_d189 = 0 mm, d204_d196_d190 = 0 mm, d205_d200_d189 = 0 mm, d440_d79 = 0 mm, d441_d80 = 0 mm, d442_d82 = 3 mm, d443_d83 = 3 mm, d444_d84 = 3 mm, d445_d85 = 3 mm, d461_d460 = 0 mm, d462_d432 = 0 mm, d463_d433 = 0 mm, d464_d434 = 0 mm, d465_d435 = 0 mm, d467_d461_d460 = 0 mm, d468_d462_d432 = 0 mm, d469_d463_d433 = 0 mm, d470_d464_d434 = 0 mm, d471_d465_d435 = 0 mm, d472_d466 = 0 mm, d474_d467_d461_d460 = 0 mm, d475_d468_d462_d432 = 0 mm, d476_d469_d463_d433 = 0 mm, d477_d470_d464_d434 = 0 mm, d478_d471_d465_d435 = 0 mm, d479_d472_d466 = 0 mm, d481_d474_d467_d461_d460 = 0 mm, d482_d475_d468_d462_d432 = 0 mm, d483_d476_d469_d463_d433 = 0 mm, d484_d477_d470_d464_d434 = 0 mm, d485_d478_d471_d465_d435 = 0 mm, d486_d479_d472_d466 = 0 mm, d488_d481_d474_d467_d461_d460 = 0 mm, d489_d482_d475_d468_d462_d432 = 0 mm, d490_d483_d476_d469_d463_d433 = 0 mm, d491_d484_d477_d470_d464_d434 = 0 mm, d492_d485_d478_d471_d465_d435 = 0 mm, d493_d486_d479_d472_d466 = 0 mm, d495_d488_d481_d474_d467_d461_d460 = 0 mm, d496_d489_d482_d475_d468_d462_d432 = 0 mm, d497_d490_d483_d476_d469_d463_d433 = 0 mm, d498_d491_d484_d477_d470_d464_d434 = 0 mm, d499_d492_d485_d478_d471_d465_d435 = 0 mm, d500_d493_d486_d479_d472_d466 = 0 mm, d502_d495_d488_d481_d474_d467_d461_d460 = 0 mm, d503_d496_d489_d482_d475_d468_d462_d432 = 0 mm, d504_d497_d490_d483_d476_d469_d463_d433 = 0 mm, d505_d498_d491_d484_d477_d470_d464_d434 = 0 mm, d506_d499_d492_d485_d478_d471_d465_d435 = 0 mm, d507_d500_d493_d486_d479_d472_d466 = 0 mm, d509_d502_d495_d488_d481_d474_d467_d461_d460 = 0 mm, d510_d503_d496_d489_d482_d475_d468_d462_d432 = 0 mm, d511_d504_d497_d490_d483_d476_d469_d463_d433 = 0 mm, d512_d505_d498_d491_d484_d477_d470_d464_d434 = 0 mm, d513_d506_d499_d492_d485_d478_d471_d465_d435 = 0 mm, d514_d507_d500_d493_d486_d479_d472_d466 = 0 mm
